# Autodesk Inventor assembly: lathe cover no ends
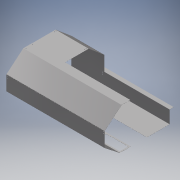
[picture p0: Inventor's stored thumbnail of the model, 180x180]
Saved by Autodesk Inventor 2016 (Build 200138000, 138)
## iProperties
Created: 2017-10-24
Part Number: lathe cover no ends
Document SubType Name: Assembly
Designer: m207653
Author: m207653
## Documents named in this file (6)
- C:\Users\m207653\Lathe with updated parts (LATEST of 20 06 17)\cover parts\Main Cover parts\lathe cover no ends.iam
- C:\Users\m207653\Lathe with updated parts (LATEST of 20 06 17)\cover parts\Main Cover parts\MC Part1.ipt
- C:\Users\m207653\Lathe with updated parts (LATEST of 20 06 17)\cover parts\Main Cover parts\MC Part2.ipt
- C:\Users\m207653\Lathe with updated parts (LATEST of 20 06 17)\cover parts\Main Cover parts\MC Part3.ipt
- C:\Users\m207653\Lathe with updated parts (LATEST of 20 06 17)\cover parts\Main Cover parts\MC Part4.ipt
- C:\Users\m207653\Lathe with updated parts (LATEST of 20 06 17)\cover parts\Main Cover parts\MC Part2b.ipt
## Components (5 placed, 5 different names)
1. MC Part1:1 — Mate:1, Rigid:5
2. MC Part2:1 — Rigid:2, Rigid:4
3. MC Part3:1 — Rigid:2, Rigid:3
4. MC Part4:1 — Rigid:3, Mate:2
5. MC Part2b:1 — Rigid:4, Rigid:5, Mate:3
## Relationships (10: WeldJoint 4, Mate 3, Angle 3)
- Rigid:2 [WeldJoint]: MC Part2:1 ↔ MC Part3:1
- Rigid:3 [WeldJoint]: MC Part3:1 ↔ MC Part4:1
- Mate:1: MC Part1:1
- Angle:1 (0 deg)
- Rigid:4 [WeldJoint]: MC Part2:1 ↔ MC Part2b:1
- Rigid:5 [WeldJoint]: MC Part1:1 ↔ MC Part2b:1
- Mate:2: MC Part4:1
- Angle:2 (0 deg)
- Mate:3: MC Part2b:1
- Angle:3 (0 deg)
